# Autodesk Inventor assembly: foot type 2 length 2
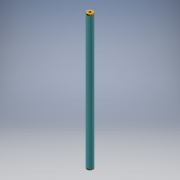
[picture p0: Inventor's stored thumbnail of the model, 180x180]
Saved by Autodesk Inventor 2018 (Build 220112000, 112)
## iProperties
Created: 2018-11-01
Part Number: foot type 2 length 2
Document SubType Name: Assembly
Designer: Admin
Author: Admin
## Documents named in this file (3)
- C:\Users\Admin\Documents\Cryostat\CAD\foot type 2 length 2.iam
- C:\Users\Admin\Documents\Cryostat\CAD\feet type 2 part 2 long.ipt
- C:\Users\Admin\Documents\Cryostat\CAD\feet type 2 part 1.ipt
## Components (3 placed, 2 different names)
1. feet type 2 part 2 long:1 — Mate:1, Mate:2, Mate:3, Mate:4
2. feet type 2 part 1:1 — Mate:1, Mate:2
3. feet type 2 part 1:2 — Mate:3, Mate:4
## Relationships (4: Mate 4)
- Mate:1: feet type 2 part 2 long:1 ↔ feet type 2 part 1:1
- Mate:2: feet type 2 part 2 long:1 ↔ feet type 2 part 1:1
- Mate:3: feet type 2 part 2 long:1 ↔ feet type 2 part 1:2
- Mate:4: feet type 2 part 2 long:1 ↔ feet type 2 part 1:2
